# Autodesk Inventor assembly: E006_Boitier_v4
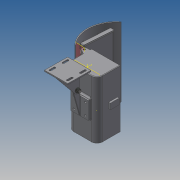
[picture p0: Inventor's stored thumbnail of the model, 180x180]
Saved by Autodesk Inventor 2021.3 (Build 253353000, 353)
## iProperties
Created: 2021-12-10
Part Number: E006_Boitier_v4
Document SubType Name: Assembly
Designer: gabri
Author: gabri
## Documents named in this file (16)
- D:\PGA\E006_Boitier_v4.iam
- D:\PGA\P037_BoitierCouvercleV4_fond.ipt
- D:\PGA\P038_BoitierCouvercleV4_couvercle.ipt
- D:\PGA\P039_BoitierCouvercleV4_capot.ipt
- D:\PGA\E003_BoitierEcran.iam
- D:\PGA\P040_BoitierCouvercleV4_module.ipt
- D:\PGA\P041_Lidar.ipt
- D:\PGA\P042_BoitierCouvercleV4_moduleHaut.ipt
- D:\PGA\P043_entretoise15par3.ipt
- C:\Users\gabri\Documents\Inventor\Content Center Files\R2021\en-US\AS 1474(2)\AS 1474 - M6(2).ipt
- D:\PGA\P044_SupportCaméra.ipt
- D:\PGA\P045_SupportUniversel.ipt
- C:\Users\gabri\Documents\Inventor\Content Center Files\R2021\en-US\ISO 4017(1)\ISO 4017 - M8 x 20 - ISO.ipt
- C:\Users\gabri\Documents\Inventor\Content Center Files\R2021\en-US\ISO 7040\DIEN EN ISO 7040 - M8.ipt
- D:\PGA\P047_BoitierCouvercleV4_porteLidar.ipt
- D:\PGA\P046_AxeCouvercleFretté.ipt
## Components (21 placed, 15 different names)
1. P037_BoitierCouvercleV4_fond:1 — Mate:1, Mate:2, Mate:3, Mate:5, Flush:2, Flush:3, Mate:10, Mate:11, Mate:12, Mate:13, Mate:20, Mate:32, Mate:33, Mate:34, Mate:35, Mate:36, Mate:37, Mate:38, Mate:39, Mate:40, Flush:4, Mate:44, Mate:58, Flush:5
2. P038_BoitierCouvercleV4_couvercle:1 — Mate:7, Mate:30, Mate:31
3. P039_BoitierCouvercleV4_capot:1 — Mate:5, Flush:2, Mate:7, Mate:30, Mate:31
4. E003_BoitierEcran:1 [sub-assembly] — Flush:3, Mate:10, Mate:11, Mate:15, Mate:16, Mate:17
5. P040_BoitierCouvercleV4_module:1 — Mate:12, Mate:13, Mate:18, Mate:19, Mate:20, Mate:21
6. P041_Lidar:1 — Mate:15, Mate:16, Mate:17
7. P042_BoitierCouvercleV4_moduleHaut:1 — Mate:18, Mate:19, Mate:21, Mate:22, Mate:23, Mate:24, Mate:25, Mate:26, Mate:27, Mate:28, Mate:29, Mate:55, Mate:56, Mate:57
8. P043_entretoise15par3:1 — Mate:22, Mate:23
9. P043_entretoise15par3:2 — Mate:24, Mate:27
10. P043_entretoise15par3:3 — Mate:25, Mate:28
11. P043_entretoise15par3:4 — Mate:26, Mate:29
12. AS 1474 (Square Nut) - Metric M6:1 — Mate:34, Mate:35
13. AS 1474 (Square Nut) - Metric M6:2 — Mate:32, Mate:33
14. AS 1474 (Square Nut) - Metric M6:3 — Mate:36, Mate:37
15. AS 1474 (Square Nut) - Metric M6:4 — Mate:38, Mate:39, Mate:41, Mate:44
16. P044_SupportCaméra:1 — Mate:40, Flush:4, Mate:41, Mate:42, Mate:43, Mate:45, Mate:46
17. P045_SupportUniversel:1 — Mate:42, Mate:43, Mate:48
18. ISO 4017 M8 x 20:1 — Mate:45, Mate:46, Mate:47
19. DIN EN ISO 7040 M8:1 — Mate:47, Mate:48
20. P047_BoitierCouvercleV4_porteLidar:1 — Mate:55, Mate:56, Mate:57
21. P046_AxeCouvercleFretté:1 — Mate:58, Flush:5
## Relationships (51: Mate 47, Flush 4)
- Mate:1: P037_BoitierCouvercleV4_fond:1
- Mate:2: P037_BoitierCouvercleV4_fond:1
- Mate:3: P037_BoitierCouvercleV4_fond:1
- Mate:5: P037_BoitierCouvercleV4_fond:1 ↔ P039_BoitierCouvercleV4_capot:1
- Flush:2: P037_BoitierCouvercleV4_fond:1 ↔ P039_BoitierCouvercleV4_capot:1
- Mate:7: P038_BoitierCouvercleV4_couvercle:1 ↔ P039_BoitierCouvercleV4_capot:1
- Flush:3: P037_BoitierCouvercleV4_fond:1 ↔ E003_BoitierEcran:1
- Mate:10: P037_BoitierCouvercleV4_fond:1 ↔ E003_BoitierEcran:1
- Mate:11: P037_BoitierCouvercleV4_fond:1 ↔ E003_BoitierEcran:1
- Mate:12: P037_BoitierCouvercleV4_fond:1 ↔ P040_BoitierCouvercleV4_module:1
- Mate:13: P037_BoitierCouvercleV4_fond:1 ↔ P040_BoitierCouvercleV4_module:1
- Mate:15 (2.75 mm): E003_BoitierEcran:1 ↔ P041_Lidar:1
- Mate:16 (0.75 mm): E003_BoitierEcran:1 ↔ P041_Lidar:1
- Mate:17 (1 mm): E003_BoitierEcran:1 ↔ P041_Lidar:1
- Mate:18: P040_BoitierCouvercleV4_module:1 ↔ P042_BoitierCouvercleV4_moduleHaut:1
- Mate:19: P040_BoitierCouvercleV4_module:1 ↔ P042_BoitierCouvercleV4_moduleHaut:1
- Mate:20: P037_BoitierCouvercleV4_fond:1 ↔ P040_BoitierCouvercleV4_module:1
- Mate:21: P040_BoitierCouvercleV4_module:1 ↔ P042_BoitierCouvercleV4_moduleHaut:1
- Mate:22: P042_BoitierCouvercleV4_moduleHaut:1 ↔ P043_entretoise15par3:1
- Mate:23: P042_BoitierCouvercleV4_moduleHaut:1 ↔ P043_entretoise15par3:1
- Mate:24: P042_BoitierCouvercleV4_moduleHaut:1 ↔ P043_entretoise15par3:2
- Mate:25: P042_BoitierCouvercleV4_moduleHaut:1 ↔ P043_entretoise15par3:3
- Mate:26: P042_BoitierCouvercleV4_moduleHaut:1 ↔ P043_entretoise15par3:4
- Mate:27: P042_BoitierCouvercleV4_moduleHaut:1 ↔ P043_entretoise15par3:2
- Mate:28: P042_BoitierCouvercleV4_moduleHaut:1 ↔ P043_entretoise15par3:3
- Mate:29: P042_BoitierCouvercleV4_moduleHaut:1 ↔ P043_entretoise15par3:4
- Mate:30: P038_BoitierCouvercleV4_couvercle:1 ↔ P039_BoitierCouvercleV4_capot:1
- Mate:31: P038_BoitierCouvercleV4_couvercle:1 ↔ P039_BoitierCouvercleV4_capot:1
- Mate:32: P037_BoitierCouvercleV4_fond:1 ↔ AS 1474 (Square Nut) - Metric M6:2
- Mate:33: P037_BoitierCouvercleV4_fond:1 ↔ AS 1474 (Square Nut) - Metric M6:2
- Mate:34: P037_BoitierCouvercleV4_fond:1 ↔ AS 1474 (Square Nut) - Metric M6:1
- Mate:35: P037_BoitierCouvercleV4_fond:1 ↔ AS 1474 (Square Nut) - Metric M6:1
- Mate:36: P037_BoitierCouvercleV4_fond:1 ↔ AS 1474 (Square Nut) - Metric M6:3
- Mate:37: P037_BoitierCouvercleV4_fond:1 ↔ AS 1474 (Square Nut) - Metric M6:3
- Mate:38: P037_BoitierCouvercleV4_fond:1 ↔ AS 1474 (Square Nut) - Metric M6:4
- Mate:39: P037_BoitierCouvercleV4_fond:1 ↔ AS 1474 (Square Nut) - Metric M6:4
- Mate:40: P037_BoitierCouvercleV4_fond:1 ↔ P044_SupportCaméra:1
- Flush:4: P037_BoitierCouvercleV4_fond:1 ↔ P044_SupportCaméra:1
- Mate:41: AS 1474 (Square Nut) - Metric M6:4 ↔ P044_SupportCaméra:1
- Mate:42: P044_SupportCaméra:1 ↔ P045_SupportUniversel:1
- Mate:43: P044_SupportCaméra:1 ↔ P045_SupportUniversel:1
- Mate:44: P037_BoitierCouvercleV4_fond:1 ↔ AS 1474 (Square Nut) - Metric M6:4
- Mate:45: P044_SupportCaméra:1 ↔ ISO 4017 M8 x 20:1
- Mate:46: P044_SupportCaméra:1 ↔ ISO 4017 M8 x 20:1
- Mate:47: ISO 4017 M8 x 20:1 ↔ DIN EN ISO 7040 M8:1
- Mate:48: P045_SupportUniversel:1 ↔ DIN EN ISO 7040 M8:1
- Mate:55: P042_BoitierCouvercleV4_moduleHaut:1 ↔ P047_BoitierCouvercleV4_porteLidar:1
- Mate:56: P042_BoitierCouvercleV4_moduleHaut:1 ↔ P047_BoitierCouvercleV4_porteLidar:1
- Mate:57: P042_BoitierCouvercleV4_moduleHaut:1 ↔ P047_BoitierCouvercleV4_porteLidar:1
- Mate:58: P037_BoitierCouvercleV4_fond:1 ↔ P046_AxeCouvercleFretté:1
- Flush:5: P037_BoitierCouvercleV4_fond:1 ↔ P046_AxeCouvercleFretté:1
